(part 1 of 2)
# Autodesk Inventor assembly: RRRC_carrier_board
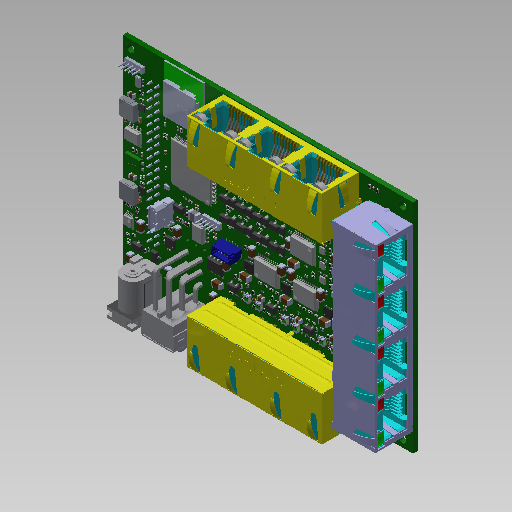
[picture p0: Inventor's stored thumbnail of the model, 512x512]
Saved by Autodesk Inventor 2019.3 (Build 233278000, 278)
## iProperties
Created: 2019-04-11
Part Number: RRRC_carrier_board
Document SubType Name: Assembly
Designer: Varga Daniel
Author: Varga Daniel
## Documents named in this file (427)
- C:\!_Dani\!_cloud\OneDrive\!_munka\Revolution\RevvyDemoKit\Structural parts\Demonstrations\Kickstarter videos\Brain pcb\RRRC_carrier_board.iam
- C:\!_Dani\!_cloud\OneDrive\!_munka\Revolution\RevvyDemoKit\Structural parts\Demonstrations\Kickstarter videos\Brain pcb\Board_CARRIER_3.iam
- C:\!_Dani\!_cloud\OneDrive\!_munka\Revolution\RevvyDemoKit\Structural parts\Demonstrations\Kickstarter videos\Brain pcb\D59_CARRIER_3.iam
- C:\!_Dani\!_cloud\OneDrive\!_munka\Revolution\RevvyDemoKit\Structural parts\Demonstrations\Kickstarter videos\Brain pcb\D15_CARRIER_3.iam
- C:\!_Dani\!_cloud\OneDrive\!_munka\Revolution\RevvyDemoKit\Structural parts\Demonstrations\Kickstarter videos\Brain pcb\C71_CARRIER_3.iam
- C:\!_Dani\!_cloud\OneDrive\!_munka\Revolution\RevvyDemoKit\Structural parts\Demonstrations\Kickstarter videos\Brain pcb\D71_CARRIER_3.iam
- C:\!_Dani\!_cloud\OneDrive\!_munka\Revolution\RevvyDemoKit\Structural parts\Demonstrations\Kickstarter videos\Brain pcb\D70_CARRIER_3.iam
- C:\!_Dani\!_cloud\OneDrive\!_munka\Revolution\RevvyDemoKit\Structural parts\Demonstrations\Kickstarter videos\Brain pcb\D69_CARRIER_3.iam
- C:\!_Dani\!_cloud\OneDrive\!_munka\Revolution\RevvyDemoKit\Structural parts\Demonstrations\Kickstarter videos\Brain pcb\D68_CARRIER_3.iam
- C:\!_Dani\!_cloud\OneDrive\!_munka\Revolution\RevvyDemoKit\Structural parts\Demonstrations\Kickstarter videos\Brain pcb\D67_CARRIER_3.iam
- C:\!_Dani\!_cloud\OneDrive\!_munka\Revolution\RevvyDemoKit\Structural parts\Demonstrations\Kickstarter videos\Brain pcb\D66_CARRIER_3.iam
- C:\!_Dani\!_cloud\OneDrive\!_munka\Revolution\RevvyDemoKit\Structural parts\Demonstrations\Kickstarter videos\Brain pcb\D65_CARRIER_3.iam
- C:\!_Dani\!_cloud\OneDrive\!_munka\Revolution\RevvyDemoKit\Structural parts\Demonstrations\Kickstarter videos\Brain pcb\D64_CARRIER_3.iam
- C:\!_Dani\!_cloud\OneDrive\!_munka\Revolution\RevvyDemoKit\Structural parts\Demonstrations\Kickstarter videos\Brain pcb\D63_CARRIER_3.iam
- C:\!_Dani\!_cloud\OneDrive\!_munka\Revolution\RevvyDemoKit\Structural parts\Demonstrations\Kickstarter videos\Brain pcb\D62_CARRIER_3.iam
- C:\!_Dani\!_cloud\OneDrive\!_munka\Revolution\RevvyDemoKit\Structural parts\Demonstrations\Kickstarter videos\Brain pcb\D61_CARRIER_3.iam
- C:\!_Dani\!_cloud\OneDrive\!_munka\Revolution\RevvyDemoKit\Structural parts\Demonstrations\Kickstarter videos\Brain pcb\D60_CARRIER_3.iam
- C:\!_Dani\!_cloud\OneDrive\!_munka\Revolution\RevvyDemoKit\Structural parts\Demonstrations\Kickstarter videos\Brain pcb\D11_CARRIER_3.iam
- C:\!_Dani\!_cloud\OneDrive\!_munka\Revolution\RevvyDemoKit\Structural parts\Demonstrations\Kickstarter videos\Brain pcb\R99_CARRIER_3.iam
- C:\!_Dani\!_cloud\OneDrive\!_munka\Revolution\RevvyDemoKit\Structural parts\Demonstrations\Kickstarter videos\Brain pcb\D58_CARRIER_3.iam
- C:\!_Dani\!_cloud\OneDrive\!_munka\Revolution\RevvyDemoKit\Structural parts\Demonstrations\Kickstarter videos\Brain pcb\D57_CARRIER_3.iam
- C:\!_Dani\!_cloud\OneDrive\!_munka\Revolution\RevvyDemoKit\Structural parts\Demonstrations\Kickstarter videos\Brain pcb\D56_CARRIER_3.iam
- C:\!_Dani\!_cloud\OneDrive\!_munka\Revolution\RevvyDemoKit\Structural parts\Demonstrations\Kickstarter videos\Brain pcb\R160_CARRIER_3.iam
- C:\!_Dani\!_cloud\OneDrive\!_munka\Revolution\RevvyDemoKit\Structural parts\Demonstrations\Kickstarter videos\Brain pcb\R159_CARRIER_3.iam
- C:\!_Dani\!_cloud\OneDrive\!_munka\Revolution\RevvyDemoKit\Structural parts\Demonstrations\Kickstarter videos\Brain pcb\R158_CARRIER_3.iam
- C:\!_Dani\!_cloud\OneDrive\!_munka\Revolution\RevvyDemoKit\Structural parts\Demonstrations\Kickstarter videos\Brain pcb\Q19_CARRIER_3.iam
- C:\!_Dani\!_cloud\OneDrive\!_munka\Revolution\RevvyDemoKit\Structural parts\Demonstrations\Kickstarter videos\Brain pcb\D24_CARRIER_3.iam
- C:\!_Dani\!_cloud\OneDrive\!_munka\Revolution\RevvyDemoKit\Structural parts\Demonstrations\Kickstarter videos\Brain pcb\CON1_CARRIER_3.iam
- C:\!_Dani\!_cloud\OneDrive\!_munka\Revolution\RevvyDemoKit\Structural parts\Demonstrations\Kickstarter videos\Brain pcb\D54_CARRIER_3.iam
- C:\!_Dani\!_cloud\OneDrive\!_munka\Revolution\RevvyDemoKit\Structural parts\Demonstrations\Kickstarter videos\Brain pcb\D55_CARRIER_3.iam
- C:\!_Dani\!_cloud\OneDrive\!_munka\Revolution\RevvyDemoKit\Structural parts\Demonstrations\Kickstarter videos\Brain pcb\Q17_CARRIER_3.iam
- C:\!_Dani\!_cloud\OneDrive\!_munka\Revolution\RevvyDemoKit\Structural parts\Demonstrations\Kickstarter videos\Brain pcb\Q18_CARRIER_3.iam
- C:\!_Dani\!_cloud\OneDrive\!_munka\Revolution\RevvyDemoKit\Structural parts\Demonstrations\Kickstarter videos\Brain pcb\R142_CARRIER_3.iam
- C:\!_Dani\!_cloud\OneDrive\!_munka\Revolution\RevvyDemoKit\Structural parts\Demonstrations\Kickstarter videos\Brain pcb\R144_CARRIER_3.iam
- C:\!_Dani\!_cloud\OneDrive\!_munka\Revolution\RevvyDemoKit\Structural parts\Demonstrations\Kickstarter videos\Brain pcb\R147_CARRIER_3.iam
- C:\!_Dani\!_cloud\OneDrive\!_munka\Revolution\RevvyDemoKit\Structural parts\Demonstrations\Kickstarter videos\Brain pcb\R139_CARRIER_3.iam
- C:\!_Dani\!_cloud\OneDrive\!_munka\Revolution\RevvyDemoKit\Structural parts\Demonstrations\Kickstarter videos\Brain pcb\R135_CARRIER_3.iam
- C:\!_Dani\!_cloud\OneDrive\!_munka\Revolution\RevvyDemoKit\Structural parts\Demonstrations\Kickstarter videos\Brain pcb\R133_CARRIER_3.iam
- C:\!_Dani\!_cloud\OneDrive\!_munka\Revolution\RevvyDemoKit\Structural parts\Demonstrations\Kickstarter videos\Brain pcb\Q16_CARRIER_3.iam
- C:\!_Dani\!_cloud\OneDrive\!_munka\Revolution\RevvyDemoKit\Structural parts\Demonstrations\Kickstarter videos\Brain pcb\Q15_CARRIER_3.iam
- C:\!_Dani\!_cloud\OneDrive\!_munka\Revolution\RevvyDemoKit\Structural parts\Demonstrations\Kickstarter videos\Brain pcb\D53_CARRIER_3.iam
- C:\!_Dani\!_cloud\OneDrive\!_munka\Revolution\RevvyDemoKit\Structural parts\Demonstrations\Kickstarter videos\Brain pcb\D52_CARRIER_3.iam
- C:\!_Dani\!_cloud\OneDrive\!_munka\Revolution\RevvyDemoKit\Structural parts\Demonstrations\Kickstarter videos\Brain pcb\D50_CARRIER_3.iam
- C:\!_Dani\!_cloud\OneDrive\!_munka\Revolution\RevvyDemoKit\Structural parts\Demonstrations\Kickstarter videos\Brain pcb\D51_CARRIER_3.iam
- C:\!_Dani\!_cloud\OneDrive\!_munka\Revolution\RevvyDemoKit\Structural parts\Demonstrations\Kickstarter videos\Brain pcb\Q13_CARRIER_3.iam
- C:\!_Dani\!_cloud\OneDrive\!_munka\Revolution\RevvyDemoKit\Structural parts\Demonstrations\Kickstarter videos\Brain pcb\Q14_CARRIER_3.iam
- C:\!_Dani\!_cloud\OneDrive\!_munka\Revolution\RevvyDemoKit\Structural parts\Demonstrations\Kickstarter videos\Brain pcb\R126_CARRIER_3.iam
- C:\!_Dani\!_cloud\OneDrive\!_munka\Revolution\RevvyDemoKit\Structural parts\Demonstrations\Kickstarter videos\Brain pcb\R127_CARRIER_3.iam
- C:\!_Dani\!_cloud\OneDrive\!_munka\Revolution\RevvyDemoKit\Structural parts\Demonstrations\Kickstarter videos\Brain pcb\R132_CARRIER_3.iam
- C:\!_Dani\!_cloud\OneDrive\!_munka\Revolution\RevvyDemoKit\Structural parts\Demonstrations\Kickstarter videos\Brain pcb\CON9_CARRIER_2.iam
- C:\!_Dani\!_cloud\OneDrive\!_munka\Revolution\RevvyDemoKit\Structural parts\Demonstrations\Kickstarter videos\Brain pcb\C42_CARRIER_3.iam
- C:\!_Dani\!_cloud\OneDrive\!_munka\Revolution\RevvyDemoKit\Structural parts\Demonstrations\Kickstarter videos\Brain pcb\C39_CARRIER_3.iam
- C:\!_Dani\!_cloud\OneDrive\!_munka\Revolution\RevvyDemoKit\Structural parts\Demonstrations\Kickstarter videos\Brain pcb\C33_CARRIER_3.iam
- C:\!_Dani\!_cloud\OneDrive\!_munka\Revolution\RevvyDemoKit\Structural parts\Demonstrations\Kickstarter videos\Brain pcb\C36_CARRIER_3.iam
- C:\!_Dani\!_cloud\OneDrive\!_munka\Revolution\RevvyDemoKit\Structural parts\Demonstrations\Kickstarter videos\Brain pcb\C86_CARRIER_3.iam
- C:\!_Dani\!_cloud\OneDrive\!_munka\Revolution\RevvyDemoKit\Structural parts\Demonstrations\Kickstarter videos\Brain pcb\C90_CARRIER_3.iam
- C:\!_Dani\!_cloud\OneDrive\!_munka\Revolution\RevvyDemoKit\Structural parts\Demonstrations\Kickstarter videos\Brain pcb\D37_CARRIER_3.iam
- C:\!_Dani\!_cloud\OneDrive\!_munka\Revolution\RevvyDemoKit\Structural parts\Demonstrations\Kickstarter videos\Brain pcb\D38_CARRIER_3.iam
- C:\!_Dani\!_cloud\OneDrive\!_munka\Revolution\RevvyDemoKit\Structural parts\Demonstrations\Kickstarter videos\Brain pcb\D42_CARRIER_3.iam
- C:\!_Dani\!_cloud\OneDrive\!_munka\Revolution\RevvyDemoKit\Structural parts\Demonstrations\Kickstarter videos\Brain pcb\D43_CARRIER_3.iam
- C:\!_Dani\!_cloud\OneDrive\!_munka\Revolution\RevvyDemoKit\Structural parts\Demonstrations\Kickstarter videos\Brain pcb\U16_CARRIER_3.iam
- C:\!_Dani\!_cloud\OneDrive\!_munka\Revolution\RevvyDemoKit\Structural parts\Demonstrations\Kickstarter videos\Brain pcb\R32_CARRIER_3.iam
- C:\!_Dani\!_cloud\OneDrive\!_munka\Revolution\RevvyDemoKit\Structural parts\Demonstrations\Kickstarter videos\Brain pcb\R40_CARRIER_3.iam
- C:\!_Dani\!_cloud\OneDrive\!_munka\Revolution\RevvyDemoKit\Structural parts\Demonstrations\Kickstarter videos\Brain pcb\R38_CARRIER_3.iam
- C:\!_Dani\!_cloud\OneDrive\!_munka\Revolution\RevvyDemoKit\Structural parts\Demonstrations\Kickstarter videos\Brain pcb\R37_CARRIER_3.iam
- C:\!_Dani\!_cloud\OneDrive\!_munka\Revolution\RevvyDemoKit\Structural parts\Demonstrations\Kickstarter videos\Brain pcb\R35_CARRIER_3.iam
- C:\!_Dani\!_cloud\OneDrive\!_munka\Revolution\RevvyDemoKit\Structural parts\Demonstrations\Kickstarter videos\Brain pcb\R34_CARRIER_3.iam
- C:\!_Dani\!_cloud\OneDrive\!_munka\Revolution\RevvyDemoKit\Structural parts\Demonstrations\Kickstarter videos\Brain pcb\R33_CARRIER_3.iam
- C:\!_Dani\!_cloud\OneDrive\!_munka\Revolution\RevvyDemoKit\Structural parts\Demonstrations\Kickstarter videos\Brain pcb\R31_CARRIER_3.iam
- C:\!_Dani\!_cloud\OneDrive\!_munka\Revolution\RevvyDemoKit\Structural parts\Demonstrations\Kickstarter videos\Brain pcb\Q5_CARRIER_3.iam
- C:\!_Dani\!_cloud\OneDrive\!_munka\Revolution\RevvyDemoKit\Structural parts\Demonstrations\Kickstarter videos\Brain pcb\FU8_CARRIER_3.iam
- C:\!_Dani\!_cloud\OneDrive\!_munka\Revolution\RevvyDemoKit\Structural parts\Demonstrations\Kickstarter videos\Brain pcb\FU7_CARRIER_3.iam
- C:\!_Dani\!_cloud\OneDrive\!_munka\Revolution\RevvyDemoKit\Structural parts\Demonstrations\Kickstarter videos\Brain pcb\D36_CARRIER_3.iam
- C:\!_Dani\!_cloud\OneDrive\!_munka\Revolution\RevvyDemoKit\Structural parts\Demonstrations\Kickstarter videos\Brain pcb\D35_CARRIER_3.iam
- C:\!_Dani\!_cloud\OneDrive\!_munka\Revolution\RevvyDemoKit\Structural parts\Demonstrations\Kickstarter videos\Brain pcb\D34_CARRIER_3.iam
- C:\!_Dani\!_cloud\OneDrive\!_munka\Revolution\RevvyDemoKit\Structural parts\Demonstrations\Kickstarter videos\Brain pcb\C63_CARRIER_3.iam
- C:\!_Dani\!_cloud\OneDrive\!_munka\Revolution\RevvyDemoKit\Structural parts\Demonstrations\Kickstarter videos\Brain pcb\C37_CARRIER_3.iam
- C:\!_Dani\!_cloud\OneDrive\!_munka\Revolution\RevvyDemoKit\Structural parts\Demonstrations\Kickstarter videos\Brain pcb\C35_CARRIER_3.iam
- C:\!_Dani\!_cloud\OneDrive\!_munka\Revolution\RevvyDemoKit\Structural parts\Demonstrations\Kickstarter videos\Brain pcb\C75_CARRIER_3.iam
- C:\!_Dani\!_cloud\OneDrive\!_munka\Revolution\RevvyDemoKit\Structural parts\Demonstrations\Kickstarter videos\Brain pcb\C77_CARRIER_3.iam
- C:\!_Dani\!_cloud\OneDrive\!_munka\Revolution\RevvyDemoKit\Structural parts\Demonstrations\Kickstarter videos\Brain pcb\C79_CARRIER_3.iam
- C:\!_Dani\!_cloud\OneDrive\!_munka\Revolution\RevvyDemoKit\Structural parts\Demonstrations\Kickstarter videos\Brain pcb\C81_CARRIER_3.iam
- C:\!_Dani\!_cloud\OneDrive\!_munka\Revolution\RevvyDemoKit\Structural parts\Demonstrations\Kickstarter videos\Brain pcb\D39_CARRIER_3.iam
- C:\!_Dani\!_cloud\OneDrive\!_munka\Revolution\RevvyDemoKit\Structural parts\Demonstrations\Kickstarter videos\Brain pcb\D40_CARRIER_3.iam
- C:\!_Dani\!_cloud\OneDrive\!_munka\Revolution\RevvyDemoKit\Structural parts\Demonstrations\Kickstarter videos\Brain pcb\D41_CARRIER_3.iam
- C:\!_Dani\!_cloud\OneDrive\!_munka\Revolution\RevvyDemoKit\Structural parts\Demonstrations\Kickstarter videos\Brain pcb\FU10_CARRIER_3.iam
- C:\!_Dani\!_cloud\OneDrive\!_munka\Revolution\RevvyDemoKit\Structural parts\Demonstrations\Kickstarter videos\Brain pcb\FU9_CARRIER_3.iam
- C:\!_Dani\!_cloud\OneDrive\!_munka\Revolution\RevvyDemoKit\Structural parts\Demonstrations\Kickstarter videos\Brain pcb\Q6_CARRIER_3.iam
- C:\!_Dani\!_cloud\OneDrive\!_munka\Revolution\RevvyDemoKit\Structural parts\Demonstrations\Kickstarter videos\Brain pcb\R36_CARRIER_3.iam
- C:\!_Dani\!_cloud\OneDrive\!_munka\Revolution\RevvyDemoKit\Structural parts\Demonstrations\Kickstarter videos\Brain pcb\R39_CARRIER_3.iam
- C:\!_Dani\!_cloud\OneDrive\!_munka\Revolution\RevvyDemoKit\Structural parts\Demonstrations\Kickstarter videos\Brain pcb\R42_CARRIER_3.iam
- C:\!_Dani\!_cloud\OneDrive\!_munka\Revolution\RevvyDemoKit\Structural parts\Demonstrations\Kickstarter videos\Brain pcb\R43_CARRIER_3.iam
- C:\!_Dani\!_cloud\OneDrive\!_munka\Revolution\RevvyDemoKit\Structural parts\Demonstrations\Kickstarter videos\Brain pcb\R44_CARRIER_3.iam
- C:\!_Dani\!_cloud\OneDrive\!_munka\Revolution\RevvyDemoKit\Structural parts\Demonstrations\Kickstarter videos\Brain pcb\R46_CARRIER_3.iam
- C:\!_Dani\!_cloud\OneDrive\!_munka\Revolution\RevvyDemoKit\Structural parts\Demonstrations\Kickstarter videos\Brain pcb\R47_CARRIER_3.iam
- C:\!_Dani\!_cloud\OneDrive\!_munka\Revolution\RevvyDemoKit\Structural parts\Demonstrations\Kickstarter videos\Brain pcb\R48_CARRIER_3.iam
- C:\!_Dani\!_cloud\OneDrive\!_munka\Revolution\RevvyDemoKit\Structural parts\Demonstrations\Kickstarter videos\Brain pcb\C32_CARRIER_3.iam
- C:\!_Dani\!_cloud\OneDrive\!_munka\Revolution\RevvyDemoKit\Structural parts\Demonstrations\Kickstarter videos\Brain pcb\C24_CARRIER_3.iam
- C:\!_Dani\!_cloud\OneDrive\!_munka\Revolution\RevvyDemoKit\Structural parts\Demonstrations\Kickstarter videos\Brain pcb\C28_CARRIER_3.iam
- C:\!_Dani\!_cloud\OneDrive\!_munka\Revolution\RevvyDemoKit\Structural parts\Demonstrations\Kickstarter videos\Brain pcb\C34_CARRIER_3.iam
- C:\!_Dani\!_cloud\OneDrive\!_munka\Revolution\RevvyDemoKit\Structural parts\Demonstrations\Kickstarter videos\Brain pcb\C73_CARRIER_3.iam
- C:\!_Dani\!_cloud\OneDrive\!_munka\Revolution\RevvyDemoKit\Structural parts\Demonstrations\Kickstarter videos\Brain pcb\D31_CARRIER_3.iam
- C:\!_Dani\!_cloud\OneDrive\!_munka\Revolution\RevvyDemoKit\Structural parts\Demonstrations\Kickstarter videos\Brain pcb\D32_CARRIER_3.iam
- C:\!_Dani\!_cloud\OneDrive\!_munka\Revolution\RevvyDemoKit\Structural parts\Demonstrations\Kickstarter videos\Brain pcb\D33_CARRIER_3.iam
- C:\!_Dani\!_cloud\OneDrive\!_munka\Revolution\RevvyDemoKit\Structural parts\Demonstrations\Kickstarter videos\Brain pcb\U15_CARRIER_3.iam
- C:\!_Dani\!_cloud\OneDrive\!_munka\Revolution\RevvyDemoKit\Structural parts\Demonstrations\Kickstarter videos\Brain pcb\U5_CARRIER_3.iam
- C:\!_Dani\!_cloud\OneDrive\!_munka\Revolution\RevvyDemoKit\Structural parts\Demonstrations\Kickstarter videos\Brain pcb\R29_CARRIER_3.iam
- C:\!_Dani\!_cloud\OneDrive\!_munka\Revolution\RevvyDemoKit\Structural parts\Demonstrations\Kickstarter videos\Brain pcb\R28_CARRIER_3.iam
- C:\!_Dani\!_cloud\OneDrive\!_munka\Revolution\RevvyDemoKit\Structural parts\Demonstrations\Kickstarter videos\Brain pcb\R24_CARRIER_3.iam
- C:\!_Dani\!_cloud\OneDrive\!_munka\Revolution\RevvyDemoKit\Structural parts\Demonstrations\Kickstarter videos\Brain pcb\R30_CARRIER_3.iam
- C:\!_Dani\!_cloud\OneDrive\!_munka\Revolution\RevvyDemoKit\Structural parts\Demonstrations\Kickstarter videos\Brain pcb\Q4_CARRIER_3.iam
- C:\!_Dani\!_cloud\OneDrive\!_munka\Revolution\RevvyDemoKit\Structural parts\Demonstrations\Kickstarter videos\Brain pcb\FU6_CARRIER_3.iam
- C:\!_Dani\!_cloud\OneDrive\!_munka\Revolution\RevvyDemoKit\Structural parts\Demonstrations\Kickstarter videos\Brain pcb\FU5_CARRIER_3.iam
- C:\!_Dani\!_cloud\OneDrive\!_munka\Revolution\RevvyDemoKit\Structural parts\Demonstrations\Kickstarter videos\Brain pcb\D14_CARRIER_3.iam
- C:\!_Dani\!_cloud\OneDrive\!_munka\Revolution\RevvyDemoKit\Structural parts\Demonstrations\Kickstarter videos\Brain pcb\D13_CARRIER_3.iam
- C:\!_Dani\!_cloud\OneDrive\!_munka\Revolution\RevvyDemoKit\Structural parts\Demonstrations\Kickstarter videos\Brain pcb\D12_CARRIER_3.iam
- C:\!_Dani\!_cloud\OneDrive\!_munka\Revolution\RevvyDemoKit\Structural parts\Demonstrations\Kickstarter videos\Brain pcb\C46_CARRIER_3.iam
- C:\!_Dani\!_cloud\OneDrive\!_munka\Revolution\RevvyDemoKit\Structural parts\Demonstrations\Kickstarter videos\Brain pcb\C53_CARRIER_3.iam
- C:\!_Dani\!_cloud\OneDrive\!_munka\Revolution\RevvyDemoKit\Structural parts\Demonstrations\Kickstarter videos\Brain pcb\C31_CARRIER_3.iam
- C:\!_Dani\!_cloud\OneDrive\!_munka\Revolution\RevvyDemoKit\Structural parts\Demonstrations\Kickstarter videos\Brain pcb\C30_CARRIER_3.iam
- C:\!_Dani\!_cloud\OneDrive\!_munka\Revolution\RevvyDemoKit\Structural parts\Demonstrations\Kickstarter videos\Brain pcb\C27_CARRIER_3.iam
- C:\!_Dani\!_cloud\OneDrive\!_munka\Revolution\RevvyDemoKit\Structural parts\Demonstrations\Kickstarter videos\Brain pcb\C29_CARRIER_3.iam
- C:\!_Dani\!_cloud\OneDrive\!_munka\Revolution\RevvyDemoKit\Structural parts\Demonstrations\Kickstarter videos\Brain pcb\R25_CARRIER_3.iam
- C:\!_Dani\!_cloud\OneDrive\!_munka\Revolution\RevvyDemoKit\Structural parts\Demonstrations\Kickstarter videos\Brain pcb\R26_CARRIER_3.iam
- C:\!_Dani\!_cloud\OneDrive\!_munka\Revolution\RevvyDemoKit\Structural parts\Demonstrations\Kickstarter videos\Brain pcb\R18_CARRIER_3.iam
- C:\!_Dani\!_cloud\OneDrive\!_munka\Revolution\RevvyDemoKit\Structural parts\Demonstrations\Kickstarter videos\Brain pcb\R17_CARRIER_3.iam
- C:\!_Dani\!_cloud\OneDrive\!_munka\Revolution\RevvyDemoKit\Structural parts\Demonstrations\Kickstarter videos\Brain pcb\C21_CARRIER_3.iam
- C:\!_Dani\!_cloud\OneDrive\!_munka\Revolution\RevvyDemoKit\Structural parts\Demonstrations\Kickstarter videos\Brain pcb\C19_CARRIER_3.iam
- C:\!_Dani\!_cloud\OneDrive\!_munka\Revolution\RevvyDemoKit\Structural parts\Demonstrations\Kickstarter videos\Brain pcb\C23_CARRIER_3.iam
- C:\!_Dani\!_cloud\OneDrive\!_munka\Revolution\RevvyDemoKit\Structural parts\Demonstrations\Kickstarter videos\Brain pcb\C25_CARRIER_3.iam
- C:\!_Dani\!_cloud\OneDrive\!_munka\Revolution\RevvyDemoKit\Structural parts\Demonstrations\Kickstarter videos\Brain pcb\C49_CARRIER_3.iam
- C:\!_Dani\!_cloud\OneDrive\!_munka\Revolution\RevvyDemoKit\Structural parts\Demonstrations\Kickstarter videos\Brain pcb\C51_CARRIER_3.iam
- C:\!_Dani\!_cloud\OneDrive\!_munka\Revolution\RevvyDemoKit\Structural parts\Demonstrations\Kickstarter videos\Brain pcb\D10_CARRIER_3.iam
- C:\!_Dani\!_cloud\OneDrive\!_munka\Revolution\RevvyDemoKit\Structural parts\Demonstrations\Kickstarter videos\Brain pcb\D8_CARRIER_3.iam
- C:\!_Dani\!_cloud\OneDrive\!_munka\Revolution\RevvyDemoKit\Structural parts\Demonstrations\Kickstarter videos\Brain pcb\D9_CARRIER_3.iam
- C:\!_Dani\!_cloud\OneDrive\!_munka\Revolution\RevvyDemoKit\Structural parts\Demonstrations\Kickstarter videos\Brain pcb\FU3_CARRIER_3.iam
- C:\!_Dani\!_cloud\OneDrive\!_munka\Revolution\RevvyDemoKit\Structural parts\Demonstrations\Kickstarter videos\Brain pcb\FU4_CARRIER_3.iam
- C:\!_Dani\!_cloud\OneDrive\!_munka\Revolution\RevvyDemoKit\Structural parts\Demonstrations\Kickstarter videos\Brain pcb\Q3_CARRIER_3.iam
- C:\!_Dani\!_cloud\OneDrive\!_munka\Revolution\RevvyDemoKit\Structural parts\Demonstrations\Kickstarter videos\Brain pcb\R11_CARRIER_3.iam
- C:\!_Dani\!_cloud\OneDrive\!_munka\Revolution\RevvyDemoKit\Structural parts\Demonstrations\Kickstarter videos\Brain pcb\R15_CARRIER_3.iam
- C:\!_Dani\!_cloud\OneDrive\!_munka\Revolution\RevvyDemoKit\Structural parts\Demonstrations\Kickstarter videos\Brain pcb\R22_CARRIER_3.iam
- C:\!_Dani\!_cloud\OneDrive\!_munka\Revolution\RevvyDemoKit\Structural parts\Demonstrations\Kickstarter videos\Brain pcb\R16_CARRIER_3.iam
- C:\!_Dani\!_cloud\OneDrive\!_munka\Revolution\RevvyDemoKit\Structural parts\Demonstrations\Kickstarter videos\Brain pcb\R20_CARRIER_3.iam
- C:\!_Dani\!_cloud\OneDrive\!_munka\Revolution\RevvyDemoKit\Structural parts\Demonstrations\Kickstarter videos\Brain pcb\R21_CARRIER_3.iam
- C:\!_Dani\!_cloud\OneDrive\!_munka\Revolution\RevvyDemoKit\Structural parts\Demonstrations\Kickstarter videos\Brain pcb\U4_CARRIER_3.iam
- C:\!_Dani\!_cloud\OneDrive\!_munka\Revolution\RevvyDemoKit\Structural parts\Demonstrations\Kickstarter videos\Brain pcb\R143_CARRIER_3.iam
- C:\!_Dani\!_cloud\OneDrive\!_munka\Revolution\RevvyDemoKit\Structural parts\Demonstrations\Kickstarter videos\Brain pcb\C82_CARRIER_3.iam
- C:\!_Dani\!_cloud\OneDrive\!_munka\Revolution\RevvyDemoKit\Structural parts\Demonstrations\Kickstarter videos\Brain pcb\C84_CARRIER_3.iam
- C:\!_Dani\!_cloud\OneDrive\!_munka\Revolution\RevvyDemoKit\Structural parts\Demonstrations\Kickstarter videos\Brain pcb\C110_CARRIER_3.iam
- C:\!_Dani\!_cloud\OneDrive\!_munka\Revolution\RevvyDemoKit\Structural parts\Demonstrations\Kickstarter videos\Brain pcb\C111_CARRIER_3.iam
- C:\!_Dani\!_cloud\OneDrive\!_munka\Revolution\RevvyDemoKit\Structural parts\Demonstrations\Kickstarter videos\Brain pcb\C112_CARRIER_3.iam
- C:\!_Dani\!_cloud\OneDrive\!_munka\Revolution\RevvyDemoKit\Structural parts\Demonstrations\Kickstarter videos\Brain pcb\D27_CARRIER_3.iam
- C:\!_Dani\!_cloud\OneDrive\!_munka\Revolution\RevvyDemoKit\Structural parts\Demonstrations\Kickstarter videos\Brain pcb\D28_CARRIER_3.iam
- C:\!_Dani\!_cloud\OneDrive\!_munka\Revolution\RevvyDemoKit\Structural parts\Demonstrations\Kickstarter videos\Brain pcb\FB7_CARRIER_3.iam
- C:\!_Dani\!_cloud\OneDrive\!_munka\Revolution\RevvyDemoKit\Structural parts\Demonstrations\Kickstarter videos\Brain pcb\FB16_CARRIER_3.iam
- C:\!_Dani\!_cloud\OneDrive\!_munka\Revolution\RevvyDemoKit\Structural parts\Demonstrations\Kickstarter videos\Brain pcb\FU19_CARRIER_3.iam
- C:\!_Dani\!_cloud\OneDrive\!_munka\Revolution\RevvyDemoKit\Structural parts\Demonstrations\Kickstarter videos\Brain pcb\FU20_CARRIER_3.iam
- C:\!_Dani\!_cloud\OneDrive\!_munka\Revolution\RevvyDemoKit\Structural parts\Demonstrations\Kickstarter videos\Brain pcb\R100_CARRIER_3.iam
- C:\!_Dani\!_cloud\OneDrive\!_munka\Revolution\RevvyDemoKit\Structural parts\Demonstrations\Kickstarter videos\Brain pcb\R101_CARRIER_3.iam
- C:\!_Dani\!_cloud\OneDrive\!_munka\Revolution\RevvyDemoKit\Structural parts\Demonstrations\Kickstarter videos\Brain pcb\R104_CARRIER_3.iam
- C:\!_Dani\!_cloud\OneDrive\!_munka\Revolution\RevvyDemoKit\Structural parts\Demonstrations\Kickstarter videos\Brain pcb\R141_CARRIER_3.iam
- C:\!_Dani\!_cloud\OneDrive\!_munka\Revolution\RevvyDemoKit\Structural parts\Demonstrations\Kickstarter videos\Brain pcb\R145_CARRIER_3.iam
- C:\!_Dani\!_cloud\OneDrive\!_munka\Revolution\RevvyDemoKit\Structural parts\Demonstrations\Kickstarter videos\Brain pcb\R146_CARRIER_3.iam
- C:\!_Dani\!_cloud\OneDrive\!_munka\Revolution\RevvyDemoKit\Structural parts\Demonstrations\Kickstarter videos\Brain pcb\D21_CARRIER_3.iam
- C:\!_Dani\!_cloud\OneDrive\!_munka\Revolution\RevvyDemoKit\Structural parts\Demonstrations\Kickstarter videos\Brain pcb\R122_CARRIER_3.iam
- C:\!_Dani\!_cloud\OneDrive\!_munka\Revolution\RevvyDemoKit\Structural parts\Demonstrations\Kickstarter videos\Brain pcb\R121_CARRIER_3.iam
- C:\!_Dani\!_cloud\OneDrive\!_munka\Revolution\RevvyDemoKit\Structural parts\Demonstrations\Kickstarter videos\Brain pcb\R89_CARRIER_3.iam
- C:\!_Dani\!_cloud\OneDrive\!_munka\Revolution\RevvyDemoKit\Structural parts\Demonstrations\Kickstarter videos\Brain pcb\R86_CARRIER_3.iam
- C:\!_Dani\!_cloud\OneDrive\!_munka\Revolution\RevvyDemoKit\Structural parts\Demonstrations\Kickstarter videos\Brain pcb\R85_CARRIER_3.iam
- C:\!_Dani\!_cloud\OneDrive\!_munka\Revolution\RevvyDemoKit\Structural parts\Demonstrations\Kickstarter videos\Brain pcb\R118_CARRIER_3.iam
- C:\!_Dani\!_cloud\OneDrive\!_munka\Revolution\RevvyDemoKit\Structural parts\Demonstrations\Kickstarter videos\Brain pcb\FU14_CARRIER_3.iam
- C:\!_Dani\!_cloud\OneDrive\!_munka\Revolution\RevvyDemoKit\Structural parts\Demonstrations\Kickstarter videos\Brain pcb\FU13_CARRIER_3.iam
- C:\!_Dani\!_cloud\OneDrive\!_munka\Revolution\RevvyDemoKit\Structural parts\Demonstrations\Kickstarter videos\Brain pcb\FB10_CARRIER_3.iam
- C:\!_Dani\!_cloud\OneDrive\!_munka\Revolution\RevvyDemoKit\Structural parts\Demonstrations\Kickstarter videos\Brain pcb\FB4_CARRIER_3.iam
- C:\!_Dani\!_cloud\OneDrive\!_munka\Revolution\RevvyDemoKit\Structural parts\Demonstrations\Kickstarter videos\Brain pcb\D19_CARRIER_3.iam
- C:\!_Dani\!_cloud\OneDrive\!_munka\Revolution\RevvyDemoKit\Structural parts\Demonstrations\Kickstarter videos\Brain pcb\D18_CARRIER_3.iam
- C:\!_Dani\!_cloud\OneDrive\!_munka\Revolution\RevvyDemoKit\Structural parts\Demonstrations\Kickstarter videos\Brain pcb\D17_CARRIER_3.iam
- C:\!_Dani\!_cloud\OneDrive\!_munka\Revolution\RevvyDemoKit\Structural parts\Demonstrations\Kickstarter videos\Brain pcb\C101_CARRIER_3.iam
- C:\!_Dani\!_cloud\OneDrive\!_munka\Revolution\RevvyDemoKit\Structural parts\Demonstrations\Kickstarter videos\Brain pcb\C99_CARRIER_3.iam
- C:\!_Dani\!_cloud\OneDrive\!_munka\Revolution\RevvyDemoKit\Structural parts\Demonstrations\Kickstarter videos\Brain pcb\C100_CARRIER_3.iam
- C:\!_Dani\!_cloud\OneDrive\!_munka\Revolution\RevvyDemoKit\Structural parts\Demonstrations\Kickstarter videos\Brain pcb\C72_CARRIER_3.iam
- C:\!_Dani\!_cloud\OneDrive\!_munka\Revolution\RevvyDemoKit\Structural parts\Demonstrations\Kickstarter videos\Brain pcb\C70_CARRIER_3.iam
- C:\!_Dani\!_cloud\OneDrive\!_munka\Revolution\RevvyDemoKit\Structural parts\Demonstrations\Kickstarter videos\Brain pcb\C74_CARRIER_3.iam
- C:\!_Dani\!_cloud\OneDrive\!_munka\Revolution\RevvyDemoKit\Structural parts\Demonstrations\Kickstarter videos\Brain pcb\C76_CARRIER_3.iam
- C:\!_Dani\!_cloud\OneDrive\!_munka\Revolution\RevvyDemoKit\Structural parts\Demonstrations\Kickstarter videos\Brain pcb\C102_CARRIER_3.iam
- C:\!_Dani\!_cloud\OneDrive\!_munka\Revolution\RevvyDemoKit\Structural parts\Demonstrations\Kickstarter videos\Brain pcb\C103_CARRIER_3.iam
- C:\!_Dani\!_cloud\OneDrive\!_munka\Revolution\RevvyDemoKit\Structural parts\Demonstrations\Kickstarter videos\Brain pcb\C105_CARRIER_3.iam
- C:\!_Dani\!_cloud\OneDrive\!_munka\Revolution\RevvyDemoKit\Structural parts\Demonstrations\Kickstarter videos\Brain pcb\D20_CARRIER_3.iam
- C:\!_Dani\!_cloud\OneDrive\!_munka\Revolution\RevvyDemoKit\Structural parts\Demonstrations\Kickstarter videos\Brain pcb\D22_CARRIER_3.iam
- C:\!_Dani\!_cloud\OneDrive\!_munka\Revolution\RevvyDemoKit\Structural parts\Demonstrations\Kickstarter videos\Brain pcb\FB5_CARRIER_3.iam
- C:\!_Dani\!_cloud\OneDrive\!_munka\Revolution\RevvyDemoKit\Structural parts\Demonstrations\Kickstarter videos\Brain pcb\FB12_CARRIER_3.iam
- C:\!_Dani\!_cloud\OneDrive\!_munka\Revolution\RevvyDemoKit\Structural parts\Demonstrations\Kickstarter videos\Brain pcb\FU15_CARRIER_3.iam
- C:\!_Dani\!_cloud\OneDrive\!_munka\Revolution\RevvyDemoKit\Structural parts\Demonstrations\Kickstarter videos\Brain pcb\FU16_CARRIER_3.iam
- C:\!_Dani\!_cloud\OneDrive\!_munka\Revolution\RevvyDemoKit\Structural parts\Demonstrations\Kickstarter videos\Brain pcb\R90_CARRIER_3.iam
- C:\!_Dani\!_cloud\OneDrive\!_munka\Revolution\RevvyDemoKit\Structural parts\Demonstrations\Kickstarter videos\Brain pcb\R91_CARRIER_3.iam
- C:\!_Dani\!_cloud\OneDrive\!_munka\Revolution\RevvyDemoKit\Structural parts\Demonstrations\Kickstarter videos\Brain pcb\R93_CARRIER_3.iam
- C:\!_Dani\!_cloud\OneDrive\!_munka\Revolution\RevvyDemoKit\Structural parts\Demonstrations\Kickstarter videos\Brain pcb\R94_CARRIER_3.iam
- C:\!_Dani\!_cloud\OneDrive\!_munka\Revolution\RevvyDemoKit\Structural parts\Demonstrations\Kickstarter videos\Brain pcb\R130_CARRIER_3.iam
- C:\!_Dani\!_cloud\OneDrive\!_munka\Revolution\RevvyDemoKit\Structural parts\Demonstrations\Kickstarter videos\Brain pcb\R131_CARRIER_3.iam
- C:\!_Dani\!_cloud\OneDrive\!_munka\Revolution\RevvyDemoKit\Structural parts\Demonstrations\Kickstarter videos\Brain pcb\CON2_CARRIER_3.iam
- C:\!_Dani\!_cloud\OneDrive\!_munka\Revolution\RevvyDemoKit\Structural parts\Demonstrations\Kickstarter videos\Brain pcb\Y1_CARRIER_3.iam
- C:\!_Dani\!_cloud\OneDrive\!_munka\Revolution\RevvyDemoKit\Structural parts\Demonstrations\Kickstarter videos\Brain pcb\U30_CARRIER_3.iam
- C:\!_Dani\!_cloud\OneDrive\!_munka\Revolution\RevvyDemoKit\Structural parts\Demonstrations\Kickstarter videos\Brain pcb\U29_CARRIER_3.iam
- C:\!_Dani\!_cloud\OneDrive\!_munka\Revolution\RevvyDemoKit\Structural parts\Demonstrations\Kickstarter videos\Brain pcb\U13_CARRIER_3.iam
- C:\!_Dani\!_cloud\OneDrive\!_munka\Revolution\RevvyDemoKit\Structural parts\Demonstrations\Kickstarter videos\Brain pcb\U27_CARRIER_3.iam
- C:\!_Dani\!_cloud\OneDrive\!_munka\Revolution\RevvyDemoKit\Structural parts\Demonstrations\Kickstarter videos\Brain pcb\U12_CARRIER_3.iam
- C:\!_Dani\!_cloud\OneDrive\!_munka\Revolution\RevvyDemoKit\Structural parts\Demonstrations\Kickstarter videos\Brain pcb\U25_CARRIER_3.iam
- C:\!_Dani\!_cloud\OneDrive\!_munka\Revolution\RevvyDemoKit\Structural parts\Demonstrations\Kickstarter videos\Brain pcb\U11_CARRIER_3.iam
- C:\!_Dani\!_cloud\OneDrive\!_munka\Revolution\RevvyDemoKit\Structural parts\Demonstrations\Kickstarter videos\Brain pcb\U10_CARRIER_3.iam
- C:\!_Dani\!_cloud\OneDrive\!_munka\Revolution\RevvyDemoKit\Structural parts\Demonstrations\Kickstarter videos\Brain pcb\U20_CARRIER_3.iam
- C:\!_Dani\!_cloud\OneDrive\!_munka\Revolution\RevvyDemoKit\Structural parts\Demonstrations\Kickstarter videos\Brain pcb\U18_CARRIER_3.iam
- C:\!_Dani\!_cloud\OneDrive\!_munka\Revolution\RevvyDemoKit\Structural parts\Demonstrations\Kickstarter videos\Brain pcb\U3_CARRIER_3.iam
- C:\!_Dani\!_cloud\OneDrive\!_munka\Revolution\RevvyDemoKit\Structural parts\Demonstrations\Kickstarter videos\Brain pcb\U14_CARRIER_3.iam
- C:\!_Dani\!_cloud\OneDrive\!_munka\Revolution\RevvyDemoKit\Structural parts\Demonstrations\Kickstarter videos\Brain pcb\U9_CARRIER_3.iam
- C:\!_Dani\!_cloud\OneDrive\!_munka\Revolution\RevvyDemoKit\Structural parts\Demonstrations\Kickstarter videos\Brain pcb\U8_CARRIER_3.iam
- C:\!_Dani\!_cloud\OneDrive\!_munka\Revolution\RevvyDemoKit\Structural parts\Demonstrations\Kickstarter videos\Brain pcb\U7_CARRIER_3.iam
- C:\!_Dani\!_cloud\OneDrive\!_munka\Revolution\RevvyDemoKit\Structural parts\Demonstrations\Kickstarter videos\Brain pcb\U6_CARRIER_3.iam
- C:\!_Dani\!_cloud\OneDrive\!_munka\Revolution\RevvyDemoKit\Structural parts\Demonstrations\Kickstarter videos\Brain pcb\U2_CARRIER_3.iam
- C:\!_Dani\!_cloud\OneDrive\!_munka\Revolution\RevvyDemoKit\Structural parts\Demonstrations\Kickstarter videos\Brain pcb\U1_CARRIER_3.iam
- C:\!_Dani\!_cloud\OneDrive\!_munka\Revolution\RevvyDemoKit\Structural parts\Demonstrations\Kickstarter videos\Brain pcb\S1_CARRIER_3.iam
- C:\!_Dani\!_cloud\OneDrive\!_munka\Revolution\RevvyDemoKit\Structural parts\Demonstrations\Kickstarter videos\Brain pcb\R157_CARRIER_3.iam
- C:\!_Dani\!_cloud\OneDrive\!_munka\Revolution\RevvyDemoKit\Structural parts\Demonstrations\Kickstarter videos\Brain pcb\R156_CARRIER_3.iam
- C:\!_Dani\!_cloud\OneDrive\!_munka\Revolution\RevvyDemoKit\Structural parts\Demonstrations\Kickstarter videos\Brain pcb\R155_CARRIER_3.iam
- C:\!_Dani\!_cloud\OneDrive\!_munka\Revolution\RevvyDemoKit\Structural parts\Demonstrations\Kickstarter videos\Brain pcb\R154_CARRIER_3.iam
- C:\!_Dani\!_cloud\OneDrive\!_munka\Revolution\RevvyDemoKit\Structural parts\Demonstrations\Kickstarter videos\Brain pcb\R153_CARRIER_3.iam
- C:\!_Dani\!_cloud\OneDrive\!_munka\Revolution\RevvyDemoKit\Structural parts\Demonstrations\Kickstarter videos\Brain pcb\R152_CARRIER_3.iam
- C:\!_Dani\!_cloud\OneDrive\!_munka\Revolution\RevvyDemoKit\Structural parts\Demonstrations\Kickstarter videos\Brain pcb\R151_CARRIER_3.iam
- C:\!_Dani\!_cloud\OneDrive\!_munka\Revolution\RevvyDemoKit\Structural parts\Demonstrations\Kickstarter videos\Brain pcb\R150_CARRIER_3.iam
- C:\!_Dani\!_cloud\OneDrive\!_munka\Revolution\RevvyDemoKit\Structural parts\Demonstrations\Kickstarter videos\Brain pcb\R149_CARRIER_3.iam
- C:\!_Dani\!_cloud\OneDrive\!_munka\Revolution\RevvyDemoKit\Structural parts\Demonstrations\Kickstarter videos\Brain pcb\R148_CARRIER_3.iam
- C:\!_Dani\!_cloud\OneDrive\!_munka\Revolution\RevvyDemoKit\Structural parts\Demonstrations\Kickstarter videos\Brain pcb\R140_CARRIER_3.iam
- C:\!_Dani\!_cloud\OneDrive\!_munka\Revolution\RevvyDemoKit\Structural parts\Demonstrations\Kickstarter videos\Brain pcb\R138_CARRIER_3.iam
- C:\!_Dani\!_cloud\OneDrive\!_munka\Revolution\RevvyDemoKit\Structural parts\Demonstrations\Kickstarter videos\Brain pcb\R137_CARRIER_3.iam
- C:\!_Dani\!_cloud\OneDrive\!_munka\Revolution\RevvyDemoKit\Structural parts\Demonstrations\Kickstarter videos\Brain pcb\R136_CARRIER_3.iam
- C:\!_Dani\!_cloud\OneDrive\!_munka\Revolution\RevvyDemoKit\Structural parts\Demonstrations\Kickstarter videos\Brain pcb\R134_CARRIER_3.iam
- C:\!_Dani\!_cloud\OneDrive\!_munka\Revolution\RevvyDemoKit\Structural parts\Demonstrations\Kickstarter videos\Brain pcb\R129_CARRIER_3.iam
- C:\!_Dani\!_cloud\OneDrive\!_munka\Revolution\RevvyDemoKit\Structural parts\Demonstrations\Kickstarter videos\Brain pcb\R128_CARRIER_3.iam
- C:\!_Dani\!_cloud\OneDrive\!_munka\Revolution\RevvyDemoKit\Structural parts\Demonstrations\Kickstarter videos\Brain pcb\R125_CARRIER_3.iam
- C:\!_Dani\!_cloud\OneDrive\!_munka\Revolution\RevvyDemoKit\Structural parts\Demonstrations\Kickstarter videos\Brain pcb\R124_CARRIER_3.iam
- C:\!_Dani\!_cloud\OneDrive\!_munka\Revolution\RevvyDemoKit\Structural parts\Demonstrations\Kickstarter videos\Brain pcb\R123_CARRIER_3.iam
- C:\!_Dani\!_cloud\OneDrive\!_munka\Revolution\RevvyDemoKit\Structural parts\Demonstrations\Kickstarter videos\Brain pcb\R120_CARRIER_3.iam
- C:\!_Dani\!_cloud\OneDrive\!_munka\Revolution\RevvyDemoKit\Structural parts\Demonstrations\Kickstarter videos\Brain pcb\R119_CARRIER_3.iam
- C:\!_Dani\!_cloud\OneDrive\!_munka\Revolution\RevvyDemoKit\Structural parts\Demonstrations\Kickstarter videos\Brain pcb\R117_CARRIER_3.iam
- C:\!_Dani\!_cloud\OneDrive\!_munka\Revolution\RevvyDemoKit\Structural parts\Demonstrations\Kickstarter videos\Brain pcb\R116_CARRIER_3.iam
- C:\!_Dani\!_cloud\OneDrive\!_munka\Revolution\RevvyDemoKit\Structural parts\Demonstrations\Kickstarter videos\Brain pcb\R115_CARRIER_3.iam
- C:\!_Dani\!_cloud\OneDrive\!_munka\Revolution\RevvyDemoKit\Structural parts\Demonstrations\Kickstarter videos\Brain pcb\R112_CARRIER_3.iam
- C:\!_Dani\!_cloud\OneDrive\!_munka\Revolution\RevvyDemoKit\Structural parts\Demonstrations\Kickstarter videos\Brain pcb\R111_CARRIER_3.iam
- C:\!_Dani\!_cloud\OneDrive\!_munka\Revolution\RevvyDemoKit\Structural parts\Demonstrations\Kickstarter videos\Brain pcb\R110_CARRIER_3.iam
- C:\!_Dani\!_cloud\OneDrive\!_munka\Revolution\RevvyDemoKit\Structural parts\Demonstrations\Kickstarter videos\Brain pcb\R109_CARRIER_3.iam
- C:\!_Dani\!_cloud\OneDrive\!_munka\Revolution\RevvyDemoKit\Structural parts\Demonstrations\Kickstarter videos\Brain pcb\R108_CARRIER_3.iam
- C:\!_Dani\!_cloud\OneDrive\!_munka\Revolution\RevvyDemoKit\Structural parts\Demonstrations\Kickstarter videos\Brain pcb\R107_CARRIER_3.iam
- C:\!_Dani\!_cloud\OneDrive\!_munka\Revolution\RevvyDemoKit\Structural parts\Demonstrations\Kickstarter videos\Brain pcb\R106_CARRIER_3.iam
- C:\!_Dani\!_cloud\OneDrive\!_munka\Revolution\RevvyDemoKit\Structural parts\Demonstrations\Kickstarter videos\Brain pcb\R105_CARRIER_3.iam
- C:\!_Dani\!_cloud\OneDrive\!_munka\Revolution\RevvyDemoKit\Structural parts\Demonstrations\Kickstarter videos\Brain pcb\R98_CARRIER_3.iam
- C:\!_Dani\!_cloud\OneDrive\!_munka\Revolution\RevvyDemoKit\Structural parts\Demonstrations\Kickstarter videos\Brain pcb\R96_CARRIER_3.iam
- C:\!_Dani\!_cloud\OneDrive\!_munka\Revolution\RevvyDemoKit\Structural parts\Demonstrations\Kickstarter videos\Brain pcb\R95_CARRIER_3.iam
- C:\!_Dani\!_cloud\OneDrive\!_munka\Revolution\RevvyDemoKit\Structural parts\Demonstrations\Kickstarter videos\Brain pcb\R87_CARRIER_3.iam
- C:\!_Dani\!_cloud\OneDrive\!_munka\Revolution\RevvyDemoKit\Structural parts\Demonstrations\Kickstarter videos\Brain pcb\R84_CARRIER_3.iam
- C:\!_Dani\!_cloud\OneDrive\!_munka\Revolution\RevvyDemoKit\Structural parts\Demonstrations\Kickstarter videos\Brain pcb\R83_CARRIER_3.iam
- C:\!_Dani\!_cloud\OneDrive\!_munka\Revolution\RevvyDemoKit\Structural parts\Demonstrations\Kickstarter videos\Brain pcb\R82_CARRIER_3.iam
- C:\!_Dani\!_cloud\OneDrive\!_munka\Revolution\RevvyDemoKit\Structural parts\Demonstrations\Kickstarter videos\Brain pcb\R81_CARRIER_3.iam
- C:\!_Dani\!_cloud\OneDrive\!_munka\Revolution\RevvyDemoKit\Structural parts\Demonstrations\Kickstarter videos\Brain pcb\R80_CARRIER_3.iam
- C:\!_Dani\!_cloud\OneDrive\!_munka\Revolution\RevvyDemoKit\Structural parts\Demonstrations\Kickstarter videos\Brain pcb\R79_CARRIER_3.iam
- C:\!_Dani\!_cloud\OneDrive\!_munka\Revolution\RevvyDemoKit\Structural parts\Demonstrations\Kickstarter videos\Brain pcb\R78_CARRIER_3.iam
- C:\!_Dani\!_cloud\OneDrive\!_munka\Revolution\RevvyDemoKit\Structural parts\Demonstrations\Kickstarter videos\Brain pcb\R77_CARRIER_3.iam
- C:\!_Dani\!_cloud\OneDrive\!_munka\Revolution\RevvyDemoKit\Structural parts\Demonstrations\Kickstarter videos\Brain pcb\R76_CARRIER_3.iam
- C:\!_Dani\!_cloud\OneDrive\!_munka\Revolution\RevvyDemoKit\Structural parts\Demonstrations\Kickstarter videos\Brain pcb\R75_CARRIER_3.iam
- C:\!_Dani\!_cloud\OneDrive\!_munka\Revolution\RevvyDemoKit\Structural parts\Demonstrations\Kickstarter videos\Brain pcb\R74_CARRIER_3.iam
- C:\!_Dani\!_cloud\OneDrive\!_munka\Revolution\RevvyDemoKit\Structural parts\Demonstrations\Kickstarter videos\Brain pcb\R73_CARRIER_3.iam
- C:\!_Dani\!_cloud\OneDrive\!_munka\Revolution\RevvyDemoKit\Structural parts\Demonstrations\Kickstarter videos\Brain pcb\R72_CARRIER_3.iam
- C:\!_Dani\!_cloud\OneDrive\!_munka\Revolution\RevvyDemoKit\Structural parts\Demonstrations\Kickstarter videos\Brain pcb\R71_CARRIER_3.iam
- C:\!_Dani\!_cloud\OneDrive\!_munka\Revolution\RevvyDemoKit\Structural parts\Demonstrations\Kickstarter videos\Brain pcb\R70_CARRIER_3.iam
- C:\!_Dani\!_cloud\OneDrive\!_munka\Revolution\RevvyDemoKit\Structural parts\Demonstrations\Kickstarter videos\Brain pcb\R69_CARRIER_3.iam
- C:\!_Dani\!_cloud\OneDrive\!_munka\Revolution\RevvyDemoKit\Structural parts\Demonstrations\Kickstarter videos\Brain pcb\R68_CARRIER_3.iam
- C:\!_Dani\!_cloud\OneDrive\!_munka\Revolution\RevvyDemoKit\Structural parts\Demonstrations\Kickstarter videos\Brain pcb\R67_CARRIER_3.iam
- C:\!_Dani\!_cloud\OneDrive\!_munka\Revolution\RevvyDemoKit\Structural parts\Demonstrations\Kickstarter videos\Brain pcb\R66_CARRIER_3.iam
- C:\!_Dani\!_cloud\OneDrive\!_munka\Revolution\RevvyDemoKit\Structural parts\Demonstrations\Kickstarter videos\Brain pcb\R65_CARRIER_3.iam
- C:\!_Dani\!_cloud\OneDrive\!_munka\Revolution\RevvyDemoKit\Structural parts\Demonstrations\Kickstarter videos\Brain pcb\R64_CARRIER_3.iam
- C:\!_Dani\!_cloud\OneDrive\!_munka\Revolution\RevvyDemoKit\Structural parts\Demonstrations\Kickstarter videos\Brain pcb\R63_CARRIER_3.iam
- C:\!_Dani\!_cloud\OneDrive\!_munka\Revolution\RevvyDemoKit\Structural parts\Demonstrations\Kickstarter videos\Brain pcb\R62_CARRIER_3.iam
- C:\!_Dani\!_cloud\OneDrive\!_munka\Revolution\RevvyDemoKit\Structural parts\Demonstrations\Kickstarter videos\Brain pcb\R61_CARRIER_3.iam
- C:\!_Dani\!_cloud\OneDrive\!_munka\Revolution\RevvyDemoKit\Structural parts\Demonstrations\Kickstarter videos\Brain pcb\R60_CARRIER_3.iam
- C:\!_Dani\!_cloud\OneDrive\!_munka\Revolution\RevvyDemoKit\Structural parts\Demonstrations\Kickstarter videos\Brain pcb\R59_CARRIER_3.iam
- C:\!_Dani\!_cloud\OneDrive\!_munka\Revolution\RevvyDemoKit\Structural parts\Demonstrations\Kickstarter videos\Brain pcb\R58_CARRIER_3.iam
- C:\!_Dani\!_cloud\OneDrive\!_munka\Revolution\RevvyDemoKit\Structural parts\Demonstrations\Kickstarter videos\Brain pcb\R57_CARRIER_3.iam
- C:\!_Dani\!_cloud\OneDrive\!_munka\Revolution\RevvyDemoKit\Structural parts\Demonstrations\Kickstarter videos\Brain pcb\R56_CARRIER_3.iam
- C:\!_Dani\!_cloud\OneDrive\!_munka\Revolution\RevvyDemoKit\Structural parts\Demonstrations\Kickstarter videos\Brain pcb\R55_CARRIER_3.iam
- C:\!_Dani\!_cloud\OneDrive\!_munka\Revolution\RevvyDemoKit\Structural parts\Demonstrations\Kickstarter videos\Brain pcb\R54_CARRIER_3.iam
- C:\!_Dani\!_cloud\OneDrive\!_munka\Revolution\RevvyDemoKit\Structural parts\Demonstrations\Kickstarter videos\Brain pcb\R53_CARRIER_3.iam
- C:\!_Dani\!_cloud\OneDrive\!_munka\Revolution\RevvyDemoKit\Structural parts\Demonstrations\Kickstarter videos\Brain pcb\R52_CARRIER_3.iam
- C:\!_Dani\!_cloud\OneDrive\!_munka\Revolution\RevvyDemoKit\Structural parts\Demonstrations\Kickstarter videos\Brain pcb\R51_CARRIER_3.iam
- C:\!_Dani\!_cloud\OneDrive\!_munka\Revolution\RevvyDemoKit\Structural parts\Demonstrations\Kickstarter videos\Brain pcb\R50_CARRIER_3.iam
- C:\!_Dani\!_cloud\OneDrive\!_munka\Revolution\RevvyDemoKit\Structural parts\Demonstrations\Kickstarter videos\Brain pcb\R49_CARRIER_3.iam
- C:\!_Dani\!_cloud\OneDrive\!_munka\Revolution\RevvyDemoKit\Structural parts\Demonstrations\Kickstarter videos\Brain pcb\R45_CARRIER_3.iam
- C:\!_Dani\!_cloud\OneDrive\!_munka\Revolution\RevvyDemoKit\Structural parts\Demonstrations\Kickstarter videos\Brain pcb\R41_CARRIER_3.iam
- C:\!_Dani\!_cloud\OneDrive\!_munka\Revolution\RevvyDemoKit\Structural parts\Demonstrations\Kickstarter videos\Brain pcb\R27_CARRIER_3.iam
- C:\!_Dani\!_cloud\OneDrive\!_munka\Revolution\RevvyDemoKit\Structural parts\Demonstrations\Kickstarter videos\Brain pcb\R23_CARRIER_3.iam
- C:\!_Dani\!_cloud\OneDrive\!_munka\Revolution\RevvyDemoKit\Structural parts\Demonstrations\Kickstarter videos\Brain pcb\R19_CARRIER_3.iam
- C:\!_Dani\!_cloud\OneDrive\!_munka\Revolution\RevvyDemoKit\Structural parts\Demonstrations\Kickstarter videos\Brain pcb\R14_CARRIER_3.iam
- C:\!_Dani\!_cloud\OneDrive\!_munka\Revolution\RevvyDemoKit\Structural parts\Demonstrations\Kickstarter videos\Brain pcb\R13_CARRIER_3.iam
- C:\!_Dani\!_cloud\OneDrive\!_munka\Revolution\RevvyDemoKit\Structural parts\Demonstrations\Kickstarter videos\Brain pcb\R12_CARRIER_3.iam
- C:\!_Dani\!_cloud\OneDrive\!_munka\Revolution\RevvyDemoKit\Structural parts\Demonstrations\Kickstarter videos\Brain pcb\R10_CARRIER_3.iam
- C:\!_Dani\!_cloud\OneDrive\!_munka\Revolution\RevvyDemoKit\Structural parts\Demonstrations\Kickstarter videos\Brain pcb\R9_CARRIER_3.iam
- C:\!_Dani\!_cloud\OneDrive\!_munka\Revolution\RevvyDemoKit\Structural parts\Demonstrations\Kickstarter videos\Brain pcb\R8_CARRIER_3.iam
- C:\!_Dani\!_cloud\OneDrive\!_munka\Revolution\RevvyDemoKit\Structural parts\Demonstrations\Kickstarter videos\Brain pcb\R7_CARRIER_3.iam
- C:\!_Dani\!_cloud\OneDrive\!_munka\Revolution\RevvyDemoKit\Structural parts\Demonstrations\Kickstarter videos\Brain pcb\R6_CARRIER_3.iam
- C:\!_Dani\!_cloud\OneDrive\!_munka\Revolution\RevvyDemoKit\Structural parts\Demonstrations\Kickstarter videos\Brain pcb\R5_CARRIER_3.iam
- C:\!_Dani\!_cloud\OneDrive\!_munka\Revolution\RevvyDemoKit\Structural parts\Demonstrations\Kickstarter videos\Brain pcb\R4_CARRIER_3.iam
- C:\!_Dani\!_cloud\OneDrive\!_munka\Revolution\RevvyDemoKit\Structural parts\Demonstrations\Kickstarter videos\Brain pcb\R3_CARRIER_3.iam
- C:\!_Dani\!_cloud\OneDrive\!_munka\Revolution\RevvyDemoKit\Structural parts\Demonstrations\Kickstarter videos\Brain pcb\R2_CARRIER_3.iam
- C:\!_Dani\!_cloud\OneDrive\!_munka\Revolution\RevvyDemoKit\Structural parts\Demonstrations\Kickstarter videos\Brain pcb\R1_CARRIER_3.iam
- C:\!_Dani\!_cloud\OneDrive\!_munka\Revolution\RevvyDemoKit\Structural parts\Demonstrations\Kickstarter videos\Brain pcb\Q12_CARRIER_3.iam
- C:\!_Dani\!_cloud\OneDrive\!_munka\Revolution\RevvyDemoKit\Structural parts\Demonstrations\Kickstarter videos\Brain pcb\Q11_CARRIER_3.iam
- C:\!_Dani\!_cloud\OneDrive\!_munka\Revolution\RevvyDemoKit\Structural parts\Demonstrations\Kickstarter videos\Brain pcb\Q10_CARRIER_3.iam
- C:\!_Dani\!_cloud\OneDrive\!_munka\Revolution\RevvyDemoKit\Structural parts\Demonstrations\Kickstarter videos\Brain pcb\Q9_CARRIER_3.iam
- C:\!_Dani\!_cloud\OneDrive\!_munka\Revolution\RevvyDemoKit\Structural parts\Demonstrations\Kickstarter videos\Brain pcb\Q8_CARRIER_3.iam
- C:\!_Dani\!_cloud\OneDrive\!_munka\Revolution\RevvyDemoKit\Structural parts\Demonstrations\Kickstarter videos\Brain pcb\Q7_CARRIER_3.iam
- C:\!_Dani\!_cloud\OneDrive\!_munka\Revolution\RevvyDemoKit\Structural parts\Demonstrations\Kickstarter videos\Brain pcb\Q2_CARRIER_3.iam
- C:\!_Dani\!_cloud\OneDrive\!_munka\Revolution\RevvyDemoKit\Structural parts\Demonstrations\Kickstarter videos\Brain pcb\Q1_CARRIER_3.iam
- C:\!_Dani\!_cloud\OneDrive\!_munka\Revolution\RevvyDemoKit\Structural parts\Demonstrations\Kickstarter videos\Brain pcb\L3_CARRIER_3.iam
- C:\!_Dani\!_cloud\OneDrive\!_munka\Revolution\RevvyDemoKit\Structural parts\Demonstrations\Kickstarter videos\Brain pcb\L2_CARRIER_3.iam
- C:\!_Dani\!_cloud\OneDrive\!_munka\Revolution\RevvyDemoKit\Structural parts\Demonstrations\Kickstarter videos\Brain pcb\L1_CARRIER_3.iam
- C:\!_Dani\!_cloud\OneDrive\!_munka\Revolution\RevvyDemoKit\Structural parts\Demonstrations\Kickstarter videos\Brain pcb\FU18_CARRIER_3.iam
- C:\!_Dani\!_cloud\OneDrive\!_munka\Revolution\RevvyDemoKit\Structural parts\Demonstrations\Kickstarter videos\Brain pcb\FU17_CARRIER_3.iam
- C:\!_Dani\!_cloud\OneDrive\!_munka\Revolution\RevvyDemoKit\Structural parts\Demonstrations\Kickstarter videos\Brain pcb\FU12_CARRIER_3.iam
- C:\!_Dani\!_cloud\OneDrive\!_munka\Revolution\RevvyDemoKit\Structural parts\Demonstrations\Kickstarter videos\Brain pcb\FU11_CARRIER_3.iam
- C:\!_Dani\!_cloud\OneDrive\!_munka\Revolution\RevvyDemoKit\Structural parts\Demonstrations\Kickstarter videos\Brain pcb\FU2_CARRIER_3.iam
- C:\!_Dani\!_cloud\OneDrive\!_munka\Revolution\RevvyDemoKit\Structural parts\Demonstrations\Kickstarter videos\Brain pcb\FU1_CARRIER_3.iam
- C:\!_Dani\!_cloud\OneDrive\!_munka\Revolution\RevvyDemoKit\Structural parts\Demonstrations\Kickstarter videos\Brain pcb\FB14_CARRIER_3.iam
- C:\!_Dani\!_cloud\OneDrive\!_munka\Revolution\RevvyDemoKit\Structural parts\Demonstrations\Kickstarter videos\Brain pcb\FB6_CARRIER_3.iam
- C:\!_Dani\!_cloud\OneDrive\!_munka\Revolution\RevvyDemoKit\Structural parts\Demonstrations\Kickstarter videos\Brain pcb\FB3_CARRIER_3.iam
- C:\!_Dani\!_cloud\OneDrive\!_munka\Revolution\RevvyDemoKit\Structural parts\Demonstrations\Kickstarter videos\Brain pcb\FB2_CARRIER_3.iam
- C:\!_Dani\!_cloud\OneDrive\!_munka\Revolution\RevvyDemoKit\Structural parts\Demonstrations\Kickstarter videos\Brain pcb\FB1_CARRIER_3.iam
- C:\!_Dani\!_cloud\OneDrive\!_munka\Revolution\RevvyDemoKit\Structural parts\Demonstrations\Kickstarter videos\Brain pcb\D49_CARRIER_3.iam
- C:\!_Dani\!_cloud\OneDrive\!_munka\Revolution\RevvyDemoKit\Structural parts\Demonstrations\Kickstarter videos\Brain pcb\D48_CARRIER_3.iam
- C:\!_Dani\!_cloud\OneDrive\!_munka\Revolution\RevvyDemoKit\Structural parts\Demonstrations\Kickstarter videos\Brain pcb\D47_CARRIER_3.iam
- C:\!_Dani\!_cloud\OneDrive\!_munka\Revolution\RevvyDemoKit\Structural parts\Demonstrations\Kickstarter videos\Brain pcb\D46_CARRIER_3.iam
- C:\!_Dani\!_cloud\OneDrive\!_munka\Revolution\RevvyDemoKit\Structural parts\Demonstrations\Kickstarter videos\Brain pcb\D45_CARRIER_3.iam
- C:\!_Dani\!_cloud\OneDrive\!_munka\Revolution\RevvyDemoKit\Structural parts\Demonstrations\Kickstarter videos\Brain pcb\D44_CARRIER_3.iam
- C:\!_Dani\!_cloud\OneDrive\!_munka\Revolution\RevvyDemoKit\Structural parts\Demonstrations\Kickstarter videos\Brain pcb\D30_CARRIER_3.iam
- C:\!_Dani\!_cloud\OneDrive\!_munka\Revolution\RevvyDemoKit\Structural parts\Demonstrations\Kickstarter videos\Brain pcb\D29_CARRIER_3.iam
- C:\!_Dani\!_cloud\OneDrive\!_munka\Revolution\RevvyDemoKit\Structural parts\Demonstrations\Kickstarter videos\Brain pcb\D25_CARRIER_3.iam
- C:\!_Dani\!_cloud\OneDrive\!_munka\Revolution\RevvyDemoKit\Structural parts\Demonstrations\Kickstarter videos\Brain pcb\D23_CARRIER_3.iam
- C:\!_Dani\!_cloud\OneDrive\!_munka\Revolution\RevvyDemoKit\Structural parts\Demonstrations\Kickstarter videos\Brain pcb\D16_CARRIER_3.iam
- C:\!_Dani\!_cloud\OneDrive\!_munka\Revolution\RevvyDemoKit\Structural parts\Demonstrations\Kickstarter videos\Brain pcb\D7_CARRIER_3.iam
- C:\!_Dani\!_cloud\OneDrive\!_munka\Revolution\RevvyDemoKit\Structural parts\Demonstrations\Kickstarter videos\Brain pcb\D6_CARRIER_3.iam
- C:\!_Dani\!_cloud\OneDrive\!_munka\Revolution\RevvyDemoKit\Structural parts\Demonstrations\Kickstarter videos\Brain pcb\D5_CARRIER_3.iam
- C:\!_Dani\!_cloud\OneDrive\!_munka\Revolution\RevvyDemoKit\Structural parts\Demonstrations\Kickstarter videos\Brain pcb\D4_CARRIER_3.iam
- C:\!_Dani\!_cloud\OneDrive\!_munka\Revolution\RevvyDemoKit\Structural parts\Demonstrations\Kickstarter videos\Brain pcb\D3_CARRIER_3.iam
- C:\!_Dani\!_cloud\OneDrive\!_munka\Revolution\RevvyDemoKit\Structural parts\Demonstrations\Kickstarter videos\Brain pcb\D2_CARRIER_3.iam
- C:\!_Dani\!_cloud\OneDrive\!_munka\Revolution\RevvyDemoKit\Structural parts\Demonstrations\Kickstarter videos\Brain pcb\D1_CARRIER_3.iam
- C:\!_Dani\!_cloud\OneDrive\!_munka\Revolution\RevvyDemoKit\Structural parts\Demonstrations\Kickstarter videos\Brain pcb\CON8_CARRIER_3.iam